# Autodesk Inventor assembly: ЛЦМК.30000.10.00.00 СБ Корпус XIAO
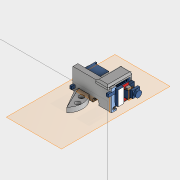
[picture p0: Inventor's stored thumbnail of the model, 180x180]
Saved by Autodesk Inventor 2021.2 (Build 252289000, 289)
## iProperties
Created: 2025-11-22
Part Number: ЛЦМК.30000.10.00.00 СБ Корпус XIAO
Document SubType Name: Assembly
Designer: Захаров
Author: Захаров
## Documents named in this file (7)
- C:\Users\User\Documents\Inventor\ЛЦМК.30000.00.00.00 Шлем\ЛЦМК.30000.10.00.00 Корпус XIAO\ЛЦМК.30000.10.00.00 СБ Корпус XIAO.iam
- C:\Users\User\Documents\Inventor\ЛЦМК.30000.00.00.00 Шлем\ЛЦМК.30000.10.00.00 Корпус XIAO\ЛЦМК.30000.10.00.04  Переходник.ipt
- C:\Users\User\Documents\Inventor\ЛЦМК.30000.00.00.00 Шлем\ЛЦМК.30000.10.00.00 Корпус XIAO\ЛЦМК.30000.10.00.01 Основание.ipt
- C:\Users\User\Documents\Inventor\ЛЦМК.30000.00.00.00 Шлем\ЛЦМК.30000.10.00.00 Корпус XIAO\XIAO.ipt
- C:\Users\User\Documents\Inventor\ЛЦМК.30000.00.00.00 Шлем\ЛЦМК.30000.10.00.00 Корпус XIAO\XIAO sense.ipt
- C:\Users\User\Documents\Inventor\ЛЦМК.30000.00.00.00 Шлем\ЛЦМК.30000.10.00.00 Корпус XIAO\ЛЦМК.30000.10.00.03 Крышка передняя.ipt
- C:\Users\User\Documents\Inventor\ЛЦМК.30000.00.00.00 Шлем\ЛЦМК.30000.10.00.00 Корпус XIAO\ЛЦМК.30000.10.00.02 Крышка задняя.ipt
## Components (6 placed, 6 different names)
1. ЛЦМК.30000.10.00.01 Основание:1 — Заподлицо:3, Совмещение:1, Совмещение:2, Заподлицо:4, Совмещение:3, Совмещение:4, Заподлицо:5, Заподлицо:6, Совмещение:8, Совмещение:9
2. ЛЦМК.30000.10.00.04  Переходник:1 — Совмещение:8, Совмещение:9
3. XIAO:1 — Заподлицо:3, Совмещение:1, Совмещение:2, Заподлицо:7
4. XIAO sense:1 — Заподлицо:4, Совмещение:3, Совмещение:4, Совмещение:5, Совмещение:6, Совмещение:7
5. ЛЦМК.30000.10.00.03 Крышка передняя:1 — Заподлицо:5, Заподлицо:6, Совмещение:5, Совмещение:6, Совмещение:7
6. ЛЦМК.30000.10.00.02 Крышка задняя:1 — Заподлицо:7
## Relationships (15: Mate 9, Flush 6)
- [Flush]: ЛЦМК.30000.10.00.01 Основание:1 ↔ ЛЦМК.30000.10.00.04  Переходник:1
- Заподлицо:3 [Flush]: ЛЦМК.30000.10.00.01 Основание:1 ↔ XIAO:1
- Совмещение:1 [Mate]: ЛЦМК.30000.10.00.01 Основание:1 ↔ XIAO:1
- Совмещение:2 [Mate]: ЛЦМК.30000.10.00.01 Основание:1 ↔ XIAO:1
- Заподлицо:4 [Flush]: ЛЦМК.30000.10.00.01 Основание:1 ↔ XIAO sense:1
- Совмещение:3 [Mate]: ЛЦМК.30000.10.00.01 Основание:1 ↔ XIAO sense:1
- Совмещение:4 [Mate]: ЛЦМК.30000.10.00.01 Основание:1 ↔ XIAO sense:1
- Заподлицо:5 [Flush]: ЛЦМК.30000.10.00.01 Основание:1 ↔ ЛЦМК.30000.10.00.03 Крышка передняя:1
- Заподлицо:6 [Flush]: ЛЦМК.30000.10.00.01 Основание:1 ↔ ЛЦМК.30000.10.00.03 Крышка передняя:1
- Совмещение:5 [Mate]: XIAO sense:1 ↔ ЛЦМК.30000.10.00.03 Крышка передняя:1
- Совмещение:6 [Mate]: XIAO sense:1 ↔ ЛЦМК.30000.10.00.03 Крышка передняя:1
- Совмещение:7 [Mate]: XIAO sense:1 ↔ ЛЦМК.30000.10.00.03 Крышка передняя:1
- Заподлицо:7 [Flush]: XIAO:1 ↔ ЛЦМК.30000.10.00.02 Крышка задняя:1
- Совмещение:8 [Mate]: ЛЦМК.30000.10.00.01 Основание:1 ↔ ЛЦМК.30000.10.00.04  Переходник:1
- Совмещение:9 [Mate]: ЛЦМК.30000.10.00.01 Основание:1 ↔ ЛЦМК.30000.10.00.04  Переходник:1
